# Autodesk Inventor assembly: 5th Wheel Hitch Fix
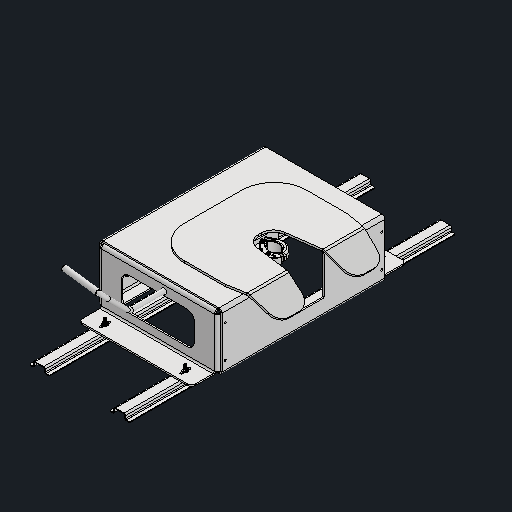
[picture p0: Inventor's stored thumbnail of the model, 512x512]
Saved by Autodesk Inventor 2025.1 (Build 291241000, 241)
## iProperties
Created: 2026-02-24
Part Number: 5th Wheel Hitch Fix
Document SubType Name: Assembly
Designer: Desktop -24
Author: Desktop -24
## Documents named in this file (10)
- F:\OneDrive - nLeague Technologies Private Limited\Desktop\Sharath Chandra\5th Wheel Hitch\5th Wheel Hitch Sliding\5th Wheel Hitch Sliding.iam
- F:\OneDrive - nLeague Technologies Private Limited\Desktop\Sharath Chandra\5th Wheel Hitch\5th Wheel Hitch Sliding\5th Wheel Hitch Sliding Part 1.ipt
- F:\OneDrive - nLeague Technologies Private Limited\Desktop\Sharath Chandra\5th Wheel Hitch\5th Wheel Hitch Sliding\5th Wheel Hitch Sliding Part 2.ipt
- F:\OneDrive - nLeague Technologies Private Limited\Desktop\Sharath Chandra\5th Wheel Hitch\5th Wheel Hitch Sliding\5th Wheel Hitch Sliding Part 3.ipt
- F:\OneDrive - nLeague Technologies Private Limited\Desktop\Sharath Chandra\5th Wheel Hitch\5th Wheel Hitch Sliding\5th Wheel Hitch Sliding Part 4.ipt
- F:\OneDrive - nLeague Technologies Private Limited\Desktop\Sharath Chandra\5th Wheel Hitch\5th Wheel Hitch Sliding\5th Wheel Hitch Sliding Part 5.ipt
- F:\OneDrive - nLeague Technologies Private Limited\Desktop\Sharath Chandra\5th Wheel Hitch\5th Wheel Hitch Sliding\5th Wheel Hitch Sliding rail.ipt
- F:\OneDrive - nLeague Technologies Private Limited\Desktop\Sharath Chandra\5th Wheel Hitch\5th Wheel Hitch Sliding\Hex Head Screw\Hex Head Screw\Hex Head Screw.ipt
- F:\OneDrive - nLeague Technologies Private Limited\Desktop\Sharath Chandra\5th Wheel Hitch\5th Wheel Hitch Sliding\Locknut\Locknut\Locknut.ipt
- F:\OneDrive - nLeague Technologies Private Limited\Desktop\Sharath Chandra\5th Wheel Hitch\5th Wheel Hitch Sliding\Washer\Washer\Washer.ipt
## Components (20 placed, 9 different names)
1. 5th Wheel Hitch Sliding Part 1:1 — Mate:1, Mate:2, Flush:1, Flush:2, Flush:3, Flush:4, Mate:3, Mate:4, Mate:5, Mate:6, Mate:7, Mate:8, Mate:9, Mate:11, Flush:5, Angle:1
2. 5th Wheel Hitch Sliding Part 2:1 — Mate:2, Flush:4, Mate:3, Flush:6
3. 5th Wheel Hitch Sliding Part 3:1 — Mate:4, Mate:6, Mate:8, Mate:10, Mate:12, Mate:14, Mate:20, Mate:21, Mate:22
4. 5th Wheel Hitch Sliding Part 3:2 — Mate:5, Mate:7, Mate:9, Mate:16
5. 5th Wheel Hitch Sliding Part 4:1 — Mate:10
6. 5th Wheel Hitch Sliding Part 5:1 — Mate:11, Flush:5, Flush:6
7. 5th Wheel Hitch Sliding rail:1 — Insert:1, Insert:2, Mate:20, Angle:1, Mate:21
8. Washer:1 — Mate:14, Mate:15
9. Locknut:1 — Mate:12, Mate:13
10. Hex Head Screw:2 — Insert:1, Mate:13, Mate:15, Mate:22
11. Locknut:2 — Mate:17, Mate:18, Mate:19
12. Washer:2 — Mate:16, Mate:17, Mate:18
13. Hex Head Screw:1 — Insert:2, Mate:19
14. 5th Wheel Hitch Sliding rail:2
15. Washer:3
16. Locknut:3
17. Hex Head Screw:3
18. Locknut:4
19. Washer:4
20. Hex Head Screw:4
## Component patterns: (2 elements, first: 5th Wheel Hitch Sliding rail:1 + Washer:1 + Locknut:1 + Hex Head Screw:2 + Locknut:2 + Washer:2 + Hex Head Screw:1)
## Relationships (31: Mate 22, Flush 6, Insert 2, Angle 1)
- Mate:1: 5th Wheel Hitch Sliding Part 1:1
- Mate:2: 5th Wheel Hitch Sliding Part 1:1 ↔ 5th Wheel Hitch Sliding Part 2:1
- Flush:1: 5th Wheel Hitch Sliding Part 1:1
- Flush:2: 5th Wheel Hitch Sliding Part 1:1
- Flush:3: 5th Wheel Hitch Sliding Part 1:1
- Flush:4: 5th Wheel Hitch Sliding Part 1:1 ↔ 5th Wheel Hitch Sliding Part 2:1
- Mate:3: 5th Wheel Hitch Sliding Part 1:1 ↔ 5th Wheel Hitch Sliding Part 2:1
- Mate:4: 5th Wheel Hitch Sliding Part 1:1 ↔ 5th Wheel Hitch Sliding Part 3:1
- Mate:5: 5th Wheel Hitch Sliding Part 1:1 ↔ 5th Wheel Hitch Sliding Part 3:2
- Mate:6: 5th Wheel Hitch Sliding Part 1:1 ↔ 5th Wheel Hitch Sliding Part 3:1
- Mate:7: 5th Wheel Hitch Sliding Part 1:1 ↔ 5th Wheel Hitch Sliding Part 3:2
- Mate:8: 5th Wheel Hitch Sliding Part 1:1 ↔ 5th Wheel Hitch Sliding Part 3:1
- Mate:9: 5th Wheel Hitch Sliding Part 1:1 ↔ 5th Wheel Hitch Sliding Part 3:2
- Mate:10: 5th Wheel Hitch Sliding Part 3:1 ↔ 5th Wheel Hitch Sliding Part 4:1
- Mate:11: 5th Wheel Hitch Sliding Part 1:1 ↔ 5th Wheel Hitch Sliding Part 5:1
- Flush:5: 5th Wheel Hitch Sliding Part 1:1 ↔ 5th Wheel Hitch Sliding Part 5:1
- Flush:6: 5th Wheel Hitch Sliding Part 2:1 ↔ 5th Wheel Hitch Sliding Part 5:1
- Insert:1: 5th Wheel Hitch Sliding rail:1 ↔ Hex Head Screw:2
- Insert:2: 5th Wheel Hitch Sliding rail:1 ↔ Hex Head Screw:1
- Mate:12: 5th Wheel Hitch Sliding Part 3:1 ↔ Locknut:1
- Mate:13: Locknut:1 ↔ Hex Head Screw:2
- Mate:14: 5th Wheel Hitch Sliding Part 3:1 ↔ Washer:1
- Mate:15: Washer:1 ↔ Hex Head Screw:2
- Mate:16: 5th Wheel Hitch Sliding Part 3:2 ↔ Washer:2
- Mate:17: Locknut:2 ↔ Washer:2
- Mate:18: Locknut:2 ↔ Washer:2
- Mate:19: Locknut:2 ↔ Hex Head Screw:1
- Mate:20: 5th Wheel Hitch Sliding Part 3:1 ↔ 5th Wheel Hitch Sliding rail:1
- Angle:1 (0 deg): 5th Wheel Hitch Sliding Part 1:1 ↔ 5th Wheel Hitch Sliding rail:1
- Mate:21: 5th Wheel Hitch Sliding Part 3:1 ↔ 5th Wheel Hitch Sliding rail:1
- Mate:22: 5th Wheel Hitch Sliding Part 3:1 ↔ Hex Head Screw:2
